# Autodesk Inventor assembly: s-assy-unit-motor
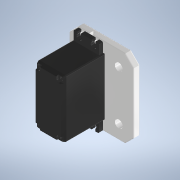
[picture p0: Inventor's stored thumbnail of the model, 180x180]
Saved by Autodesk Inventor 2022 (Build 260153000, 153)
## iProperties
Created: 2022-06-14
Part Number: s-assy-unit-motor
Document SubType Name: Assembly
Designer: yuto6
Author: yuto6
## Documents named in this file (3)
- C:\Users\yuto6\Documents\CAD\book-reader\s-assy-unit-motor-R.iam
- C:\Users\yuto6\Documents\CAD\book-reader\MG_996R.iam
- C:\Users\yuto6\Documents\CAD\book-reader\base1.ipt
## Components (2 placed, 2 different names)
1. MG_996R:1 [sub-assembly] — メイト:1, メイト:2, メイト:3
2. base1:1 — メイト:1, メイト:2, メイト:3
## Relationships (3: Mate 3)
- メイト:1 [Mate]: MG_996R:1 ↔ base1:1
- メイト:2 [Mate]: MG_996R:1 ↔ base1:1
- メイト:3 [Mate]: MG_996R:1 ↔ base1:1
